# Autodesk Inventor assembly: Pulleyschraube_80mm
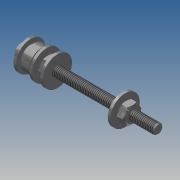
[picture p0: Inventor's stored thumbnail of the model, 180x180]
Saved by Autodesk Inventor 2015 SP1 (Build 190203100, 203)
## iProperties
Created: 2015-03-05
Part Number: Pulleyschraube_80mm
Document SubType Name: Assembly
Designer: Marc
Author: Marc
## Documents named in this file (6)
- E:\Modellflieger\3D Drucker\Eigene Teile\Eigene Schrauben\Pulleyschraube_80mm.iam
- E:\Modellflieger\3D Drucker\Eigene Teile\Eigene Schrauben\DIN 84 - M6 x 80.ipt
- E:\Modellflieger\3D Drucker\Eigene Teile\Kugellager_6x15x5_696ZZ.ipt
- C:\Users\Marc\Documents\Inventor\Content Center Files\R2015\de-DE\DIN 9021\DIN 9021 - 6,4.ipt
- C:\Users\Marc\Documents\Inventor\Content Center Files\R2015\de-DE\DIN 125-1  A\DIN 125 - A 6,4.ipt
- C:\Users\Marc\Documents\Inventor\Content Center Files\R2015\de-DE\DIN 934\DIN 934 - M6 x 1.ipt
## Components (10 placed, 5 different names)
1. DIN 84 - M6 x 80:1 — Einfügen:7, Passend:3
2. Kugellager_6x15x5_696ZZ:1
3. DIN 9021 6,4:1
4. DIN 9021 6,4:2
5. DIN 125-1 A A 6,4:1
6. DIN 125-1 A A 6,4:2
7. DIN 934 - ersetzt durch DIN EN 24032/28673/28674 M6:1
8. DIN 9021 6,4:3
9. DIN 9021 6,4:4 — Einfügen:7, Passend:4
10. DIN 934 - ersetzt durch DIN EN 24032/28673/28674 M6:2 — Passend:3, Passend:4
## Relationships (11: Insert 7, Mate 4)
- [Insert]: DIN 84 - M6 x 80:1 ↔ DIN 9021 6,4:1
- [Insert]: Kugellager_6x15x5_696ZZ:1 ↔ DIN 125-1 A A 6,4:1
- [Insert]: DIN 9021 6,4:1 ↔ DIN 125-1 A A 6,4:1
- [Insert]: Kugellager_6x15x5_696ZZ:1 ↔ DIN 125-1 A A 6,4:2
- [Insert]: DIN 9021 6,4:2 ↔ DIN 125-1 A A 6,4:2
- [Mate]: DIN 84 - M6 x 80:1 ↔ DIN 934 - ersetzt durch DIN EN 24032/28673/28674 M6:1
- [Mate]: DIN 9021 6,4:2 ↔ DIN 934 - ersetzt durch DIN EN 24032/28673/28674 M6:1
- [Insert]: DIN 934 - ersetzt durch DIN EN 24032/28673/28674 M6:1 ↔ DIN 9021 6,4:3
- Einfügen:7 [Insert] (-22 mm): DIN 84 - M6 x 80:1 ↔ DIN 9021 6,4:4
- Passend:3 [Mate]: DIN 84 - M6 x 80:1 ↔ DIN 934 - ersetzt durch DIN EN 24032/28673/28674 M6:2
- Passend:4 [Mate]: DIN 9021 6,4:4 ↔ DIN 934 - ersetzt durch DIN EN 24032/28673/28674 M6:2
## Named parameters: d381_d348_d341 = 0 mm, d382_d349_d342 = 0 mm, d383_d350_d343 = 0 mm, d384_d351_d344 = 0 mm, d385_d352_d345 = 0 mm, d386_d353_d346 = 0 mm, d387_d354_d347 = 0 mm, d388_d355 = 0 mm
